# Autodesk Inventor assembly: End Effector Platform
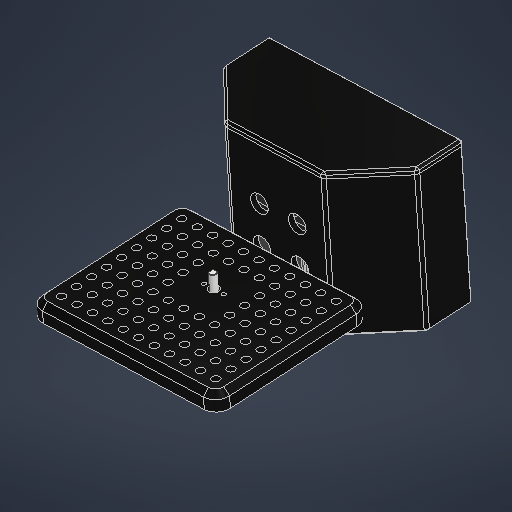
[picture p0: Inventor's stored thumbnail of the model, 512x512]
Saved by Autodesk Inventor 2026.1 (Build 301233000, 233)
## iProperties
Created: 2025-07-17
Part Number: End Effector Platform
Document SubType Name: Assembly
Designer: AdminForWorker
Title: End Effector Platform v38
Author: AdminForWorker
## Documents named in this file (8)
- C:\Users\Oasis\Documents\Work\ENGINEER 1P13 IAI Position (2024 - 2025)\P1 QArm Revamp\End Effector Platform\End Effector Platform.iam
- C:\Users\Oasis\Documents\Work\ENGINEER 1P13 IAI Position (2024 - 2025)\P1 QArm Revamp\End Effector Platform\N20 Mini Micro Metall Gear Motor DC 3-6-12V v1 v1.ipt
- C:\Users\Oasis\Documents\Work\ENGINEER 1P13 IAI Position (2024 - 2025)\P1 QArm Revamp\End Effector Platform\XC-430_idle v3.iam
- C:\Users\Oasis\Documents\Work\ENGINEER 1P13 IAI Position (2024 - 2025)\P1 QArm Revamp\End Effector Platform\End Effector Platform Base.ipt
- C:\Users\Oasis\Documents\Work\ENGINEER 1P13 IAI Position (2024 - 2025)\P1 QArm Revamp\End Effector Platform\Quanser QUARC EE Board.ipt
- C:\Users\Oasis\Documents\Work\ENGINEER 1P13 IAI Position (2024 - 2025)\P1 QArm Revamp\End Effector Platform\End Effector Platform.ipt
- C:\Users\Oasis\Documents\Work\ENGINEER 1P13 IAI Position (2024 - 2025)\P1 QArm Revamp\End Effector Platform\End Effector Platform Compartment Lid.ipt
- C:\Users\Oasis\Documents\Work\ENGINEER 1P13 IAI Position (2024 - 2025)\P1 QArm Revamp\End Effector Platform\Gripper Motor Cover.ipt
## Components (7 placed, 7 different names)
1. N20 Mini Micro Metall Gear Motor DC 3-6-12V v1 v1:1 — Flush:3, Mate:8, Mate:9, Mate:10, Mate:11, Mate:12
2. XC-430_idle v3:1 [sub-assembly] — Mate:4, Mate:5, Mate:6
3. End Effector Platform Base:1 — Mate:1, Mate:2, Mate:3, Mate:4, Mate:5, Mate:6, Flush:1, Flush:2, Mate:7, Flush:3, Mate:8, Mate:9
4. Quanser QUARC EE Board:1 — Mate:1, Mate:2, Mate:3
5. End Effector Platform:1 — Mate:10, Mate:11, Mate:12, Mate:13, Flush:4, Flush:5
6. End Effector Platform Compartment Lid:1 — Flush:1, Flush:2, Mate:7
7. Gripper Motor Cover:1 — Mate:13, Flush:4, Flush:5
## Relationships (18: Mate 13, Flush 5)
- Mate:1: End Effector Platform Base:1 ↔ Quanser QUARC EE Board:1
- Mate:2: End Effector Platform Base:1 ↔ Quanser QUARC EE Board:1
- Mate:3: End Effector Platform Base:1 ↔ Quanser QUARC EE Board:1
- Mate:4: XC-430_idle v3:1 ↔ End Effector Platform Base:1
- Mate:5: XC-430_idle v3:1 ↔ End Effector Platform Base:1
- Mate:6: XC-430_idle v3:1 ↔ End Effector Platform Base:1
- Flush:1: End Effector Platform Base:1 ↔ End Effector Platform Compartment Lid:1
- Flush:2: End Effector Platform Base:1 ↔ End Effector Platform Compartment Lid:1
- Mate:7: End Effector Platform Base:1 ↔ End Effector Platform Compartment Lid:1
- Flush:3: N20 Mini Micro Metall Gear Motor DC 3-6-12V v1 v1:1 ↔ End Effector Platform Base:1
- Mate:8 (0.2 mm): N20 Mini Micro Metall Gear Motor DC 3-6-12V v1 v1:1 ↔ End Effector Platform Base:1
- Mate:9 (0.2 mm): N20 Mini Micro Metall Gear Motor DC 3-6-12V v1 v1:1 ↔ End Effector Platform Base:1
- Mate:10: N20 Mini Micro Metall Gear Motor DC 3-6-12V v1 v1:1 ↔ End Effector Platform:1
- Mate:11: N20 Mini Micro Metall Gear Motor DC 3-6-12V v1 v1:1 ↔ End Effector Platform:1
- Mate:12: N20 Mini Micro Metall Gear Motor DC 3-6-12V v1 v1:1 ↔ End Effector Platform:1
- Mate:13: End Effector Platform:1 ↔ Gripper Motor Cover:1
- Flush:4: End Effector Platform:1 ↔ Gripper Motor Cover:1
- Flush:5: End Effector Platform:1 ↔ Gripper Motor Cover:1
